# Autodesk Inventor assembly: Test stand and ignitor
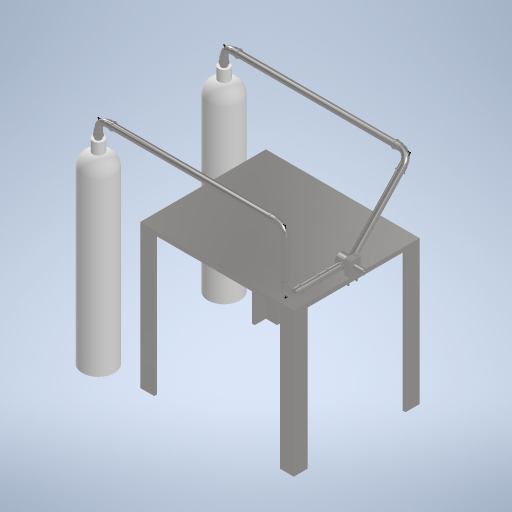
[picture p0: Inventor's stored thumbnail of the model, 512x512]
Saved by Autodesk Inventor 2024 (Build 280153020, 153B)
## iProperties
Created: 2023-08-29
Part Number: Test stand and ignitor
Document SubType Name: Assembly
Designer: Victoria
Author: Victoria
## Documents named in this file (8)
- D:\Cad cam\Final Year\Test stand and ignitor.iam
- D:\Cad cam\Final Year\Work table.ipt
- D:\Cad cam\Final Year\Cylinder.ipt
- D:\Cad cam\Final Year\Bolt.ipt
- D:\Cad cam\Final Year\Clamp.ipt
- D:\Cad cam\Final Year\ASI Propane.ipt
- C:\Users\Valentine\Documents\Inventor\Content Center Files\R2024\en-US\AS 1112 (2)\AS 1112 - M5  Type 5.ipt
- D:\Cad cam\Final Year\Test stand and ignitor.Tube and Pipe Runs.iam
## Components (11 placed, 7 different names)
1. Work table:1 — Mate:1, Mate:2, Mate:3, Mate:4, Mate:5, Mate:6, Mate:7, Insert:1, Insert:2, Insert:8, Insert:9
2. Cylinder:1 — Mate:6, Mate:7
3. Cylinder:2 — Mate:4, Mate:5
4. Bolt:1 — Insert:7
5. Bolt:2 — Insert:6
6. Clamp:1 — Insert:1, Insert:2, Insert:3, Insert:4, Insert:5, Mate:8
7. Clamp:2 — Insert:3, Insert:4, Insert:6, Insert:7
8. ASI Propane:1 — Insert:5, Mate:8
9. AS 1112 (2) - Metric M5  Type 5:1 — Insert:8
10. AS 1112 (2) - Metric M5  Type 5:2 — Insert:9
11. Tube & Pipe Runs [sub-assembly]
## Relationships (17: Insert 9, Mate 8)
- Mate:1: Work table:1
- Mate:2: Work table:1
- Mate:3: Work table:1
- Mate:4 (200 mm): Work table:1 ↔ Cylinder:2
- Mate:5: Work table:1 ↔ Cylinder:2
- Mate:6 (200 mm): Work table:1 ↔ Cylinder:1
- Mate:7: Work table:1 ↔ Cylinder:1
- Insert:1: Work table:1 ↔ Clamp:1
- Insert:2: Work table:1 ↔ Clamp:1
- Insert:3: Clamp:1 ↔ Clamp:2
- Insert:4: Clamp:1 ↔ Clamp:2
- Insert:5: Clamp:1 ↔ ASI Propane:1
- Mate:8: Clamp:1 ↔ ASI Propane:1
- Insert:6: Bolt:2 ↔ Clamp:2
- Insert:7: Bolt:1 ↔ Clamp:2
- Insert:8: Work table:1 ↔ AS 1112 (2) - Metric M5  Type 5:1
- Insert:9: Work table:1 ↔ AS 1112 (2) - Metric M5  Type 5:2
